# Autodesk Inventor assembly: Tribo_Trolly_Final
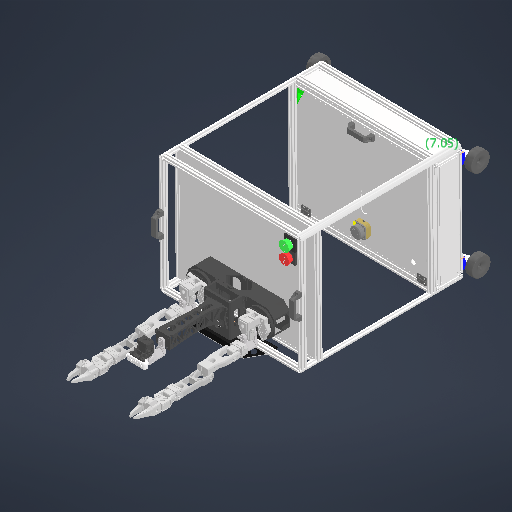
[picture p0: Inventor's stored thumbnail of the model, 512x512]
Saved by Autodesk Inventor 2026.2 (Build 302298010, 298A)
## iProperties
Created: 2026-06-10
Part Number: Tribo_Trolly_Final
Document SubType Name: Assembly
Designer: dalbi
Author: dalbi
## Documents named in this file (12)
- C:\Users\User\Desktop\트리보 관련 자료\최종 설계 파일(조립시 참고할 파일)\Tribo_Trolly_withArm.iam
- C:\Users\User\Desktop\트리보 관련 자료\최종 설계 파일(조립시 참고할 파일)\구동부_어셈블.iam
- C:\Users\User\Desktop\트리보 관련 자료\최종 설계 파일(조립시 참고할 파일)\외곽프레임.iam
- C:\Users\User\Desktop\트리보 관련 자료\최종 설계 파일(조립시 참고할 파일)\AL_Plate_Outer_600X500X2t.ipt
- C:\Users\User\Desktop\트리보 관련 자료\최종 설계 파일(조립시 참고할 파일)\multiblock_12x12x14.ipt
- C:\Users\User\Desktop\트리보 관련 자료\최종 설계 파일(조립시 참고할 파일)\Handle.ipt
- C:\Users\User\Desktop\트리보 관련 자료\최종 설계 파일(조립시 참고할 파일)\STOP_BUTTON_GREEN.ipt
- C:\Users\User\Desktop\트리보 관련 자료\최종 설계 파일(조립시 참고할 파일)\STOP_BUTTON_RED.ipt
- C:\Users\User\Desktop\트리보 관련 자료\1차설계파일\Tribo_Upper_Robot_Assy.iam
- C:\Users\User\Desktop\트리보 관련 자료\step\LCD_Mount_20degrees_V3.ipt
- C:\Users\User\Desktop\트리보 관련 자료\step\LCD_Upper_Cover.ipt
- C:\Users\User\Desktop\트리보 관련 자료\최종 설계 파일(조립시 참고할 파일)\LCD_Bottom_Cover.ipt
## Components (17 placed, 11 different names)
1. 구동부_어셈블:1 [sub-assembly] — 메이트:1, 플러쉬:1, 메이트:2
2. 외곽프레임:1 [sub-assembly] — 메이트:1, 플러쉬:1, 메이트:2, 메이트:3, 메이트:4, 플러쉬:2, 메이트:5, 플러쉬:3, 메이트:6, 메이트:7, 플러쉬:4, 메이트:8, 메이트:9, 메이트:10, 플러쉬:5, 메이트:11, 플러쉬:6, 메이트:12, 메이트:13, 플러쉬:7, 메이트:14, 메이트:16, 메이트:17, 메이트:18, 메이트:19, 플러쉬:8, 메이트:20, 플러쉬:22, 메이트:21, 메이트:31, 메이트:32, 메이트:34, 메이트:35, 메이트:41, 플러쉬:30, 메이트:42
3. AL_Plate_Outer_600X500X2t:1 — 메이트:15, 메이트:16, 메이트:17, 메이트:30, 메이트:33
4. multiblock_12x12x14:1 — 메이트:13, 플러쉬:7, 메이트:14, 메이트:15
5. multiblock_12x12x14:2 — 메이트:9, 메이트:10, 플러쉬:5
6. multiblock_12x12x14:3 — 메이트:3, 메이트:4, 플러쉬:2
7. multiblock_12x12x14:4 — 메이트:5, 플러쉬:3, 메이트:6
8. multiblock_12x12x14:5 — 메이트:7, 플러쉬:4, 메이트:8
9. multiblock_12x12x14:6 — 메이트:11, 플러쉬:6, 메이트:12
10. Handle:1 — 메이트:20, 플러쉬:22, 메이트:21
11. Handle:2 — 메이트:18, 메이트:19, 플러쉬:8
12. STOP_BUTTON_GREEN:1 — 메이트:29, 플러쉬:24, 플러쉬:25, 메이트:32
13. STOP_BUTTON_RED:1 — 메이트:29, 플러쉬:24, 플러쉬:25, 메이트:30, 메이트:31
14. Tribo_Upper_Robot_Assy:1 [sub-assembly] — 메이트:33, 메이트:34, 메이트:35
15. LCD_Mount_20degrees_V3:1 — 메이트:38, 메이트:39, 플러쉬:27, 메이트:41, 플러쉬:30, 메이트:42
16. LCD_Upper_Cover:1 — 메이트:40, 플러쉬:28, 플러쉬:29
17. LCD_Bottom_Cover:1 — 메이트:38, 메이트:39, 플러쉬:27, 메이트:40, 플러쉬:28, 플러쉬:29
## Relationships (48: Mate 33, Flush 15)
- 메이트:1 [Mate]: 구동부_어셈블:1 ↔ 외곽프레임:1
- 플러쉬:1 [Flush]: 구동부_어셈블:1 ↔ 외곽프레임:1
- 메이트:2 [Mate]: 구동부_어셈블:1 ↔ 외곽프레임:1
- 메이트:3 [Mate]: 외곽프레임:1 ↔ multiblock_12x12x14:3
- 메이트:4 [Mate]: 외곽프레임:1 ↔ multiblock_12x12x14:3
- 플러쉬:2 [Flush] (3 mm): 외곽프레임:1 ↔ multiblock_12x12x14:3
- 메이트:5 [Mate]: 외곽프레임:1 ↔ multiblock_12x12x14:4
- 플러쉬:3 [Flush] (3 mm): 외곽프레임:1 ↔ multiblock_12x12x14:4
- 메이트:6 [Mate]: 외곽프레임:1 ↔ multiblock_12x12x14:4
- 메이트:7 [Mate]: 외곽프레임:1 ↔ multiblock_12x12x14:5
- 플러쉬:4 [Flush] (3 mm): 외곽프레임:1 ↔ multiblock_12x12x14:5
- 메이트:8 [Mate] (243 mm): 외곽프레임:1 ↔ multiblock_12x12x14:5
- 메이트:9 [Mate]: 외곽프레임:1 ↔ multiblock_12x12x14:2
- 메이트:10 [Mate]: 외곽프레임:1 ↔ multiblock_12x12x14:2
- 플러쉬:5 [Flush] (-3 mm): 외곽프레임:1 ↔ multiblock_12x12x14:2
- 메이트:11 [Mate]: 외곽프레임:1 ↔ multiblock_12x12x14:6
- 플러쉬:6 [Flush] (3 mm): 외곽프레임:1 ↔ multiblock_12x12x14:6
- 메이트:12 [Mate] (243 mm): 외곽프레임:1 ↔ multiblock_12x12x14:6
- 메이트:13 [Mate]: 외곽프레임:1 ↔ multiblock_12x12x14:1
- 플러쉬:7 [Flush] (3 mm): 외곽프레임:1 ↔ multiblock_12x12x14:1
- 메이트:14 [Mate]: 외곽프레임:1 ↔ multiblock_12x12x14:1
- 메이트:15 [Mate]: AL_Plate_Outer_600X500X2t:1 ↔ multiblock_12x12x14:1
- 메이트:16 [Mate]: 외곽프레임:1 ↔ AL_Plate_Outer_600X500X2t:1
- 메이트:17 [Mate]: 외곽프레임:1 ↔ AL_Plate_Outer_600X500X2t:1
- 메이트:18 [Mate]: 외곽프레임:1 ↔ Handle:2
- 메이트:19 [Mate] (196 mm): 외곽프레임:1 ↔ Handle:2
- 플러쉬:8 [Flush] (1 mm): 외곽프레임:1 ↔ Handle:2
- 메이트:20 [Mate]: 외곽프레임:1 ↔ Handle:1
- 플러쉬:22 [Flush] (1 mm): 외곽프레임:1 ↔ Handle:1
- 메이트:21 [Mate] (196 mm): 외곽프레임:1 ↔ Handle:1
- 메이트:29 [Mate]: STOP_BUTTON_GREEN:1 ↔ STOP_BUTTON_RED:1
- 플러쉬:24 [Flush]: STOP_BUTTON_GREEN:1 ↔ STOP_BUTTON_RED:1
- 플러쉬:25 [Flush]: STOP_BUTTON_GREEN:1 ↔ STOP_BUTTON_RED:1
- 메이트:30 [Mate]: AL_Plate_Outer_600X500X2t:1 ↔ STOP_BUTTON_RED:1
- 메이트:31 [Mate] (50 mm): 외곽프레임:1 ↔ STOP_BUTTON_RED:1
- 메이트:32 [Mate] (50 mm): 외곽프레임:1 ↔ STOP_BUTTON_GREEN:1
- 메이트:33 [Mate]: AL_Plate_Outer_600X500X2t:1 ↔ Tribo_Upper_Robot_Assy:1
- 메이트:34 [Mate] (10 mm): 외곽프레임:1 ↔ Tribo_Upper_Robot_Assy:1
- 메이트:35 [Mate] (106.3 mm): 외곽프레임:1 ↔ Tribo_Upper_Robot_Assy:1
- 메이트:38 [Mate]: LCD_Mount_20degrees_V3:1 ↔ LCD_Bottom_Cover:1
- 메이트:39 [Mate]: LCD_Mount_20degrees_V3:1 ↔ LCD_Bottom_Cover:1
- 플러쉬:27 [Flush]: LCD_Mount_20degrees_V3:1 ↔ LCD_Bottom_Cover:1
- 메이트:40 [Mate]: LCD_Upper_Cover:1 ↔ LCD_Bottom_Cover:1
- 플러쉬:28 [Flush]: LCD_Upper_Cover:1 ↔ LCD_Bottom_Cover:1
- 플러쉬:29 [Flush]: LCD_Upper_Cover:1 ↔ LCD_Bottom_Cover:1
- 메이트:41 [Mate]: 외곽프레임:1 ↔ LCD_Mount_20degrees_V3:1
- 플러쉬:30 [Flush]: 외곽프레임:1 ↔ LCD_Mount_20degrees_V3:1
- 메이트:42 [Mate] (260 mm): 외곽프레임:1 ↔ LCD_Mount_20degrees_V3:1
